# Autodesk Inventor assembly: THROTTLE BODY
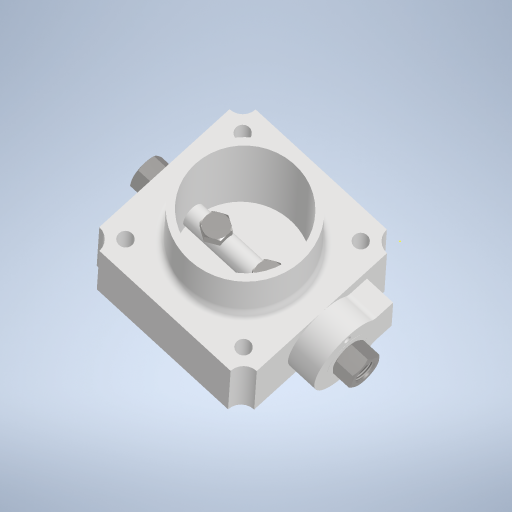
[picture p0: Inventor's stored thumbnail of the model, 512x512]
Saved by Autodesk Inventor 2023 (Build 270158000, 158)
## iProperties
Created: 2023-07-26
Part Number: THROTTLE BODY
Document SubType Name: Assembly
Designer: User
Author: User
## Documents named in this file (5)
- C:\Users\User\Desktop\BIANCA\SCHOOL WORK\INVENTOR 2023\CRUISE CONTROL\THROTTLE BODY.iam
- C:\Users\User\Desktop\BIANCA\SCHOOL WORK\INVENTOR 2023\CRUISE CONTROL\Base.ipt
- C:\Users\User\Desktop\BIANCA\SCHOOL WORK\INVENTOR 2023\CRUISE CONTROL\TPS.iam
- C:\Users\User\Desktop\BIANCA\SCHOOL WORK\INVENTOR 2023\CRUISE CONTROL\ANSI B18.2.4.2M - M14x2 - 21.ipt
- C:\Users\User\Desktop\BIANCA\SCHOOL WORK\INVENTOR 2023\CRUISE CONTROL\Throttle.iam
## Components (5 placed, 4 different names)
1. Base:1 — Rotational:1, Rigid:1, Rigid:2
2. TPS:1 [sub-assembly] — Insert:6, Rigid:2
3. ANSI B18.2.4.2M - M14x2 - 21:1 — Rigid:1
4. ANSI B18.2.4.2M - M14x2 - 21:2 — Insert:6
5. Throttle:1 [sub-assembly] — Rotational:1
## Relationships (4: WeldJoint 2, Insert 1, RevoluteJoint 1)
- Insert:6: TPS:1 ↔ ANSI B18.2.4.2M - M14x2 - 21:2
- Rotational:1 [RevoluteJoint] (-30 mm): Base:1 ↔ Throttle:1
- Rigid:1 [WeldJoint]: Base:1 ↔ ANSI B18.2.4.2M - M14x2 - 21:1
- Rigid:2 [WeldJoint]: Base:1 ↔ TPS:1
